# Autodesk Inventor assembly: CartesianRobotWorkSpace
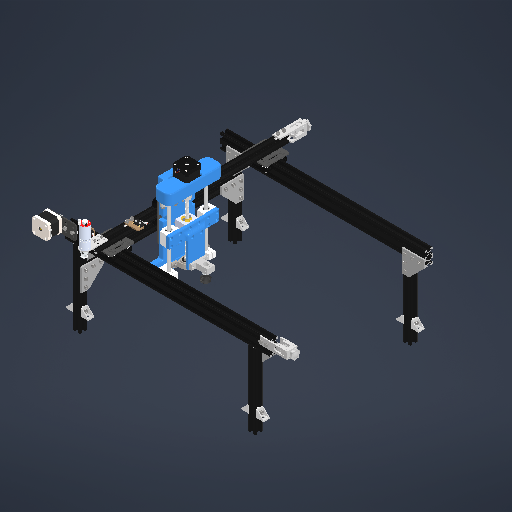
[picture p0: Inventor's stored thumbnail of the model, 512x512]
Saved by Autodesk Inventor 2027.1 (Build 311270010, 270A)
## iProperties
Created: 2026-09-29
Part Number: CartesianRobotWorkSpace
Document SubType Name: Assembly
Designer: SDS Scholar
Author: SDS Scholar
## Documents named in this file (24)
- E:\Apps\AutodeskInventor\University\MCT333_Design_of_Mechatronics_Systems_1\CAD\cartesian_robot_workspace\CartesianRobotWorkSpace.iam
- E:\Apps\AutodeskInventor\University\MCT333_Design_of_Mechatronics_Systems_1\CAD\off_the_shelf_components\AluminiumExtrusion\AluminiumExtrusion2020\Pillars.ipt
- E:\Apps\AutodeskInventor\University\MCT333_Design_of_Mechatronics_Systems_1\CAD\off_the_shelf_components\CornerBracket2020\CornerBracket2020.ipt
- C:\Users\SDS Scholar\Documents\Inventor\Content Center Files\R2027\en-US\SS-ISO 4762\ISO 4762 - M5 x 10SS-ISO.ipt
- E:\Apps\AutodeskInventor\University\MCT333_Design_of_Mechatronics_Systems_1\CAD\off_the_shelf_components\T_nuts\Slider T-Nut for 2020 - M5.ipt
- E:\Apps\AutodeskInventor\University\MCT333_Design_of_Mechatronics_Systems_1\CAD\off_the_shelf_components\RightAngleCornerPlate2020\2020 corner joining plate v1.ipt
- E:\Apps\AutodeskInventor\University\MCT333_Design_of_Mechatronics_Systems_1\CAD\off_the_shelf_components\AluminiumExtrusion\Extrusion2040\2040extrusion_ipt\X_Axis.ipt
- E:\Apps\AutodeskInventor\University\MCT333_Design_of_Mechatronics_Systems_1\CAD\off_the_shelf_components\AluminiumExtrusion\AluminiumExtrusion2020\SupportBeam.ipt
- E:\Apps\AutodeskInventor\University\MCT333_Design_of_Mechatronics_Systems_1\CAD\off_the_shelf_components\VSoltGantrySetAllSizes\20mm Gantry Set\20mm Gantry Set.ipt
- E:\Apps\AutodeskInventor\University\MCT333_Design_of_Mechatronics_Systems_1\CAD\off_the_shelf_components\RightAngleCornerPlate2020\2020 corner joining plate v1_MIR2.ipt
- E:\Apps\AutodeskInventor\University\MCT333_Design_of_Mechatronics_Systems_1\CAD\off_the_shelf_components\T_nuts\Slider T-Nut for 2020 - M5_MIR2.ipt
- E:\Apps\AutodeskInventor\University\MCT333_Design_of_Mechatronics_Systems_1\CAD\off_the_shelf_components\nema-17-23-stepper-motor-mounts\NEMA 17 Flat.ipt
- E:\Apps\AutodeskInventor\University\MCT333_Design_of_Mechatronics_Systems_1\CAD\off_the_shelf_components\GT2BeltTensioner\2020 Belt Tensioner G_K.ipt
- E:\Apps\AutodeskInventor\University\MCT333_Design_of_Mechatronics_Systems_1\CAD\cartesian_robot_workspace\Y_Axis.iam
- E:\Apps\AutodeskInventor\University\MCT333_Design_of_Mechatronics_Systems_1\CAD\cartesian_robot_workspace\Z Axis\Z-Axis.iam
- E:\Apps\AutodeskInventor\University\MCT333_Design_of_Mechatronics_Systems_1\CAD\cartesian_robot_workspace\LimitSwitchMountPlate.ipt
- E:\Apps\AutodeskInventor\University\MCT333_Design_of_Mechatronics_Systems_1\CAD\off_the_shelf_components\T_nuts\Slider T-Nut for 2020 - M3.ipt
- E:\Apps\AutodeskInventor\University\MCT333_Design_of_Mechatronics_Systems_1\CAD\electronic_components\NO-NC Bump Switch\NO-NC Bump Switch.ipt
- C:\Users\SDS Scholar\Documents\Inventor\Content Center Files\R2027\en-US\DIN 7985 (H)\DIN 7985 (H) - M2.5x12-H.ipt
- C:\Users\SDS Scholar\Documents\Inventor\Content Center Files\R2027\en-US\ISO 4032(2)\ISO 4032 - M2.5 - ISO.ipt
- C:\Users\SDS Scholar\Documents\Inventor\Content Center Files\R2027\en-US\ISO 7046-1 H(1)\ISO 7046-1 - M3 x 6_ - 4.8 - H - ISO.ipt
- E:\Apps\AutodeskInventor\University\MCT333_Design_of_Mechatronics_Systems_1\CAD\motors_and_actuators\nema17_stepper_motor\Nema17\Nema17.ipt
- E:\Apps\AutodeskInventor\University\MCT333_Design_of_Mechatronics_Systems_1\CAD\off_the_shelf_components\gt2_pulley_6\GT2 Pulley Assembly With Grub Screws\GT2 Pulley Assembly With Grub Screws.ipt
- E:\Apps\AutodeskInventor\University\MCT333_Design_of_Mechatronics_Systems_1\CAD\DESIGN1_CAD_parameters.xlsx
## Components (131 placed, 22 different names)
1. Z-Axis:1 [sub-assembly] — Tangent:9, Tangent:10, Mate:231, Mate:232
2. SupportBeam:1 — Mate:123, Mate:124, Mate:125, Mate:126, Mate:138, Mate:141, Mate:143, Mate:202
3. X_Axis:1 — Mate:32, Mate:33, Mate:34, Mate:35, Mate:36, Mate:37, Mate:48, Mate:49, Mate:56, Mate:59, Flush:3, Tangent:1, Tangent:2, Mate:145, Mate:146, Mate:147, Mate:148, Mate:151, Mate:154, Flush:6, Mate:156, Mate:157, Mate:158, Mate:159, Mate:162, Mate:165, Mate:217, Flush:193, Mate:234, Mate:235, Mate:236, Mate:237, Mate:240, Mate:243, Mate:268, Mate:271, Mate:274
4. X_Axis:2 — Mate:89, Mate:90, Mate:91, Mate:92, Mate:93, Mate:94, Mate:107, Mate:110, Mate:113, Mate:115, Flush:4, Tangent:5, Tangent:6, Mate:225
5. NEMA 17 Flat:1 — Mate:266, Mate:267, Mate:268, Mate:284, Mate:285, Mate:287, Mate:288, Mate:290, Mate:292, Mate:293, Mate:294, Mate:295, Mate:296
6. Slider T-Nut for 2020 - M5:40 — Mate:145, Mate:146, Mate:150, Flush:6
7. Slider T-Nut for 2020 - M5:41 — Mate:147, Mate:148, Mate:153
8. SS ISO 4762 M5 x 10:58 — Mate:150, Mate:151, Mate:270
9. SS ISO 4762 M5 x 10:59 — Mate:153, Mate:154, Mate:269
10. ISO 7046-1 H M3 x 6 - 4.8 - H:1 — Mate:285, Mate:286, Mate:293
11. ISO 7046-1 H M3 x 6 - 4.8 - H:2 — Mate:287, Mate:294
12. ISO 7046-1 H M3 x 6 - 4.8 - H:3 — Mate:288, Mate:289, Mate:292
13. Nema17:1 — Mate:284, Mate:286, Mate:289, Mate:291, Mate:296, Mate:297, Mate:298
14. ISO 7046-1 H M3 x 6 - 4.8 - H:4 — Mate:290, Mate:291, Mate:295
15. GT2 Pulley Assembly With Grub Screws:1 — Mate:297, Mate:298
16. 2020 Belt Tensioner G_K:1 — Mate:269, Mate:270, Mate:271
17. Slider T-Nut for 2020 - M5:42 — Mate:156, Mate:157, Mate:161, Mate:179, Flush:193
18. Slider T-Nut for 2020 - M5:43 — Mate:158, Mate:159, Mate:164
19. SS ISO 4762 M5 x 10:60 — Mate:164, Mate:165, Mate:266
20. SS ISO 4762 M5 x 10:61 — Mate:161, Mate:162, Mate:179, Mate:267
21. 20mm Gantry Set:1 — Tangent:1, Tangent:2, Flush:5, Mate:171, Flush:9, Mate:229, Mate:230
22. 20mm Gantry Set:2 — Tangent:5, Tangent:6, Flush:5, Mate:174, Mate:177, Flush:8, Flush:9
23. Y_Axis:1 [sub-assembly] — Mate:167, Mate:168, Mate:169, Mate:170, Mate:173, Mate:176, Mate:177, Flush:8, Tangent:9, Tangent:10, Mate:231, Mate:232
24. Slider T-Nut for 2020 - M5:44 — Mate:167, Mate:168, Mate:172
25. Slider T-Nut for 2020 - M5:45 — Mate:169, Mate:170, Mate:175
26. SS ISO 4762 M5 x 10:62 — Mate:174, Mate:175, Mate:176
27. SS ISO 4762 M5 x 10:63 — Mate:171, Mate:172, Mate:173
28. NO-NC Bump Switch:1 — Mate:279, Mate:280, Mate:281, Mate:282, Mate:283
29. LimitSwitchMountPlate:1 — Mate:272, Mate:273, Mate:274, Flush:194, Mate:275, Mate:276, Mate:277, Mate:278, Mate:281
30. Slider T-Nut for 2020 - M3:1 — Mate:234, Mate:235, Mate:239
31. Slider T-Nut for 2020 - M3:2 — Mate:236, Mate:237, Mate:242
32. SS ISO 4762 M5 x 10:70 — Mate:239, Mate:240, Mate:273
33. SS ISO 4762 M5 x 10:71 — Mate:242, Mate:243, Mate:272
34. DIN 7985 (H) M2.5x12-H:1 — Mate:251, Mate:275, Mate:279, Mate:282
35. DIN 7985 (H) M2.5x12-H:2 — Mate:253, Mate:276, Mate:280, Mate:283
36. ISO 4032 M2.5:1 — Mate:251, Mate:277
37. ISO 4032 M2.5:2 — Mate:253, Mate:278
38. Pillars:1 — Flush:10, Flush:11, Mate:183, Mate:184, Mate:185, Mate:186, Mate:187, Mate:188, Mate:189, Flush:191, Flush:192, Mate:190, Symmetry:1, Mate:191, Mate:192, Mate:193, Mate:194, Mate:195, Mate:196, Mate:197, Mate:198, Mate:199, Mate:200, Mate:201, Mate:202
39. SS ISO 4762 M5 x 10:2 — Mate:28, Mate:29, Mate:189
40. Slider T-Nut for 2020 - M5:2 — Mate:29, Mate:186, Mate:187
41. Slider T-Nut for 2020 - M5:1 — Mate:21, Mate:184, Mate:185
42. SS ISO 4762 M5 x 10:1 — Mate:20, Mate:21, Mate:31, Mate:188
43. CornerBracket2020:1 — Mate:20, Mate:31, Flush:191
44. CornerBracket2020:4 — Mate:28, Flush:192, Mate:190
45. Pillars:2 — Mate:218, Mate:219, Mate:220, Mate:221, Mate:222, Mate:223, Mate:224, Mate:225
46. SS ISO 4762 M5 x 10:64
47. Slider T-Nut for 2020 - M5:46
48. Slider T-Nut for 2020 - M5:47
49. SS ISO 4762 M5 x 10:65
50. CornerBracket2020:5
51. CornerBracket2020:6
52. Pillars:3 — Symmetry:1
53. SS ISO 4762 M5 x 10:66
54. Slider T-Nut for 2020 - M5:48
55. Slider T-Nut for 2020 - M5:49
56. SS ISO 4762 M5 x 10:67
57. CornerBracket2020:7
58. CornerBracket2020:8
59. Pillars:4 — Mate:210, Mate:211, Mate:212, Mate:213, Mate:214, Mate:215, Mate:216, Mate:217
60. SS ISO 4762 M5 x 10:68
61. Slider T-Nut for 2020 - M5:50
62. Slider T-Nut for 2020 - M5:51
63. SS ISO 4762 M5 x 10:69
64. CornerBracket2020:9
65. CornerBracket2020:10
66. 2020 corner joining plate v1:6 — Mate:127, Mate:130, Mate:133, Mate:136, Mate:139, Mate:143, Mate:144, Mate:201
67. Slider T-Nut for 2020 - M5:35 — Mate:131, Mate:192, Mate:195
68. Slider T-Nut for 2020 - M5:36 — Mate:123, Mate:124, Mate:137
69. Slider T-Nut for 2020 - M5:37 — Mate:134, Mate:191, Mate:194, Mate:196
70. Slider T-Nut for 2020 - M5:38 — Mate:125, Mate:126, Mate:140
71. Slider T-Nut for 2020 - M5:39 — Mate:128, Mate:193, Mate:197
72. SS ISO 4762 M5 x 10:48 — Mate:127, Mate:128, Mate:198
73. SS ISO 4762 M5 x 10:49 — Mate:139, Mate:140, Mate:141
74. SS ISO 4762 M5 x 10:50 — Mate:130, Mate:131, Mate:199
75. SS ISO 4762 M5 x 10:51 — Mate:133, Mate:134, Mate:200
76. SS ISO 4762 M5 x 10:52 — Mate:136, Mate:137, Mate:138
77. 2020 corner joining plate v1_MIR2:1
78. Slider T-Nut for 2020 - M5_MIR2:1
79. Slider T-Nut for 2020 - M5_MIR2:2
80. Slider T-Nut for 2020 - M5_MIR2:3
81. Slider T-Nut for 2020 - M5_MIR2:4
82. Slider T-Nut for 2020 - M5_MIR2:5
83. SS ISO 4762 M5 x 10:53
84. SS ISO 4762 M5 x 10:54
85. SS ISO 4762 M5 x 10:55
86. SS ISO 4762 M5 x 10:56
87. SS ISO 4762 M5 x 10:57
88. 2020 corner joining plate v1:1 — Mate:42, Mate:46, Mate:49, Mate:51, Mate:54, Mate:57, Flush:3, Mate:216, Mate:230
89. Slider T-Nut for 2020 - M5:9 — Mate:36, Mate:37, Mate:55
90. Slider T-Nut for 2020 - M5:10 — Mate:52, Mate:212, Mate:213
91. Slider T-Nut for 2020 - M5:11 — Mate:43, Mate:210, Mate:211
92. Slider T-Nut for 2020 - M5:12 — Mate:34, Mate:35, Mate:58
93. Slider T-Nut for 2020 - M5:13 — Mate:32, Mate:33, Mate:47
94. SS ISO 4762 M5 x 10:9 — Mate:42, Mate:43, Mate:215
95. SS ISO 4762 M5 x 10:10 — Mate:46, Mate:47, Mate:48
96. SS ISO 4762 M5 x 10:11 — Mate:54, Mate:55, Mate:56
97. SS ISO 4762 M5 x 10:12 — Mate:51, Mate:52, Mate:214
98. SS ISO 4762 M5 x 10:13 — Mate:57, Mate:58, Mate:59
99. 2020 corner joining plate v1:2 — Mate:229, Flush:194
100. Slider T-Nut for 2020 - M5:14
101. Slider T-Nut for 2020 - M5:15
102. Slider T-Nut for 2020 - M5:16
103. Slider T-Nut for 2020 - M5:17
104. Slider T-Nut for 2020 - M5:18
105. SS ISO 4762 M5 x 10:14
106. SS ISO 4762 M5 x 10:15
107. SS ISO 4762 M5 x 10:16
108. SS ISO 4762 M5 x 10:17
109. SS ISO 4762 M5 x 10:18
110. 2020 corner joining plate v1:4 — Mate:99, Mate:102, Mate:105, Mate:108, Mate:111, Mate:115, Flush:4, Mate:224
111. Slider T-Nut for 2020 - M5:25 — Mate:93, Mate:94, Mate:106
112. Slider T-Nut for 2020 - M5:26 — Mate:103, Mate:218, Mate:219
113. Slider T-Nut for 2020 - M5:27 — Mate:100, Mate:220, Mate:221
114. Slider T-Nut for 2020 - M5:28 — Mate:91, Mate:92, Mate:109
115. Slider T-Nut for 2020 - M5:29 — Mate:89, Mate:90, Mate:112
116. SS ISO 4762 M5 x 10:38 — Mate:99, Mate:100, Mate:223
117. SS ISO 4762 M5 x 10:39 — Mate:105, Mate:106, Mate:107
118. SS ISO 4762 M5 x 10:40 — Mate:102, Mate:103, Mate:222
119. SS ISO 4762 M5 x 10:41 — Mate:108, Mate:109, Mate:110
120. SS ISO 4762 M5 x 10:42 — Mate:111, Mate:112, Mate:113
121. 2020 corner joining plate v1:5 — Mate:144
122. Slider T-Nut for 2020 - M5:30
123. Slider T-Nut for 2020 - M5:31
124. Slider T-Nut for 2020 - M5:32
125. Slider T-Nut for 2020 - M5:33
126. Slider T-Nut for 2020 - M5:34
127. SS ISO 4762 M5 x 10:43
128. SS ISO 4762 M5 x 10:44
129. SS ISO 4762 M5 x 10:45
130. SS ISO 4762 M5 x 10:46
131. SS ISO 4762 M5 x 10:47
## Component patterns: (4 elements, first: Pillars:1 + SS ISO 4762 M5 x 10:2 + Slider T-Nut for 2020 - M5:2 + Slider T-Nut for 2020 - M5:1 + SS ISO 4762 M5 x 10:1 + CornerBracket2020:1 + CornerBracket2020:4), (2 elements, first: 2020 corner joining plate v1:6 + Slider T-Nut for 2020 - M5:35 + Slider T-Nut for 2020 - M5:36 + Slider T-Nut for 2020 - M5:37 + Slider T-Nut for 2020 - M5:38 + Slider T-Nut for 2020 - M5:39 + SS ISO 4762 M5 x 10:48 + SS ISO 4762 M5 x 10:49 + SS ISO 4762 M5 x 10:50 + SS ISO 4762 M5 x 10:51 + SS ISO 4762 M5 x 10:52), (2 elements, first: 2020 corner joining plate v1:1 + Slider T-Nut for 2020 - M5:9 + Slider T-Nut for 2020 - M5:10 + Slider T-Nut for 2020 - M5:11 + Slider T-Nut for 2020 - M5:12 + Slider T-Nut for 2020 - M5:13 + SS ISO 4762 M5 x 10:9 + SS ISO 4762 M5 x 10:10 + SS ISO 4762 M5 x 10:11 + SS ISO 4762 M5 x 10:12 + SS ISO 4762 M5 x 10:13), (2 elements, first: 2020 corner joining plate v1:4 + Slider T-Nut for 2020 - M5:25 + Slider T-Nut for 2020 - M5:26 + Slider T-Nut for 2020 - M5:27 + Slider T-Nut for 2020 - M5:28 + Slider T-Nut for 2020 - M5:29 + SS ISO 4762 M5 x 10:38 + SS ISO 4762 M5 x 10:39 + SS ISO 4762 M5 x 10:40 + SS ISO 4762 M5 x 10:41 + SS ISO 4762 M5 x 10:42)
## Relationships (193: Mate 174, Flush 12, Tangent 6, Symmetry 1)
- Mate:20: SS ISO 4762 M5 x 10:1 ↔ CornerBracket2020:1
- Mate:21: Slider T-Nut for 2020 - M5:1 ↔ SS ISO 4762 M5 x 10:1
- Mate:28: SS ISO 4762 M5 x 10:2 ↔ CornerBracket2020:4
- Mate:29: SS ISO 4762 M5 x 10:2 ↔ Slider T-Nut for 2020 - M5:2
- Mate:31 (0.7 mm): SS ISO 4762 M5 x 10:1 ↔ CornerBracket2020:1
- Mate:32: X_Axis:1 ↔ Slider T-Nut for 2020 - M5:13
- Mate:33: X_Axis:1 ↔ Slider T-Nut for 2020 - M5:13
- Mate:34: X_Axis:1 ↔ Slider T-Nut for 2020 - M5:12
- Mate:35: X_Axis:1 ↔ Slider T-Nut for 2020 - M5:12
- Mate:36: X_Axis:1 ↔ Slider T-Nut for 2020 - M5:9
- Mate:37: X_Axis:1 ↔ Slider T-Nut for 2020 - M5:9
- Mate:42: 2020 corner joining plate v1:1 ↔ SS ISO 4762 M5 x 10:9
- Mate:43: Slider T-Nut for 2020 - M5:11 ↔ SS ISO 4762 M5 x 10:9
- Mate:46: 2020 corner joining plate v1:1 ↔ SS ISO 4762 M5 x 10:10
- Mate:47: Slider T-Nut for 2020 - M5:13 ↔ SS ISO 4762 M5 x 10:10
- Mate:48: X_Axis:1 ↔ SS ISO 4762 M5 x 10:10
- Mate:49: X_Axis:1 ↔ 2020 corner joining plate v1:1
- Mate:51: 2020 corner joining plate v1:1 ↔ SS ISO 4762 M5 x 10:12
- Mate:52: Slider T-Nut for 2020 - M5:10 ↔ SS ISO 4762 M5 x 10:12
- Mate:54: 2020 corner joining plate v1:1 ↔ SS ISO 4762 M5 x 10:11
- Mate:55: Slider T-Nut for 2020 - M5:9 ↔ SS ISO 4762 M5 x 10:11
- Mate:56: X_Axis:1 ↔ SS ISO 4762 M5 x 10:11
- Mate:57: 2020 corner joining plate v1:1 ↔ SS ISO 4762 M5 x 10:13
- Mate:58: Slider T-Nut for 2020 - M5:12 ↔ SS ISO 4762 M5 x 10:13
- Mate:59: X_Axis:1 ↔ SS ISO 4762 M5 x 10:13
- Flush:3: X_Axis:1 ↔ 2020 corner joining plate v1:1
- Tangent:1: X_Axis:1 ↔ 20mm Gantry Set:1
- Tangent:2: X_Axis:1 ↔ 20mm Gantry Set:1
- Mate:89: X_Axis:2 ↔ Slider T-Nut for 2020 - M5:29
- Mate:90: X_Axis:2 ↔ Slider T-Nut for 2020 - M5:29
- Mate:91: X_Axis:2 ↔ Slider T-Nut for 2020 - M5:28
- Mate:92: X_Axis:2 ↔ Slider T-Nut for 2020 - M5:28
- Mate:93: X_Axis:2 ↔ Slider T-Nut for 2020 - M5:25
- Mate:94: X_Axis:2 ↔ Slider T-Nut for 2020 - M5:25
- Mate:99: 2020 corner joining plate v1:4 ↔ SS ISO 4762 M5 x 10:38
- Mate:100: Slider T-Nut for 2020 - M5:27 ↔ SS ISO 4762 M5 x 10:38
- Mate:102: 2020 corner joining plate v1:4 ↔ SS ISO 4762 M5 x 10:40
- Mate:103: Slider T-Nut for 2020 - M5:26 ↔ SS ISO 4762 M5 x 10:40
- Mate:105: 2020 corner joining plate v1:4 ↔ SS ISO 4762 M5 x 10:39
- Mate:106: Slider T-Nut for 2020 - M5:25 ↔ SS ISO 4762 M5 x 10:39
- Mate:107: X_Axis:2 ↔ SS ISO 4762 M5 x 10:39
- Mate:108: 2020 corner joining plate v1:4 ↔ SS ISO 4762 M5 x 10:41
- Mate:109: Slider T-Nut for 2020 - M5:28 ↔ SS ISO 4762 M5 x 10:41
- Mate:110: X_Axis:2 ↔ SS ISO 4762 M5 x 10:41
- Mate:111: 2020 corner joining plate v1:4 ↔ SS ISO 4762 M5 x 10:42
- Mate:112: Slider T-Nut for 2020 - M5:29 ↔ SS ISO 4762 M5 x 10:42
- Mate:113: X_Axis:2 ↔ SS ISO 4762 M5 x 10:42
- Mate:115: X_Axis:2 ↔ 2020 corner joining plate v1:4
- Flush:4: X_Axis:2 ↔ 2020 corner joining plate v1:4
- Mate:123: SupportBeam:1 ↔ Slider T-Nut for 2020 - M5:36
- Mate:124: SupportBeam:1 ↔ Slider T-Nut for 2020 - M5:36
- Mate:125: SupportBeam:1 ↔ Slider T-Nut for 2020 - M5:38
- Mate:126: SupportBeam:1 ↔ Slider T-Nut for 2020 - M5:38
- Mate:127: 2020 corner joining plate v1:6 ↔ SS ISO 4762 M5 x 10:48
- Mate:128: Slider T-Nut for 2020 - M5:39 ↔ SS ISO 4762 M5 x 10:48
- Mate:130: 2020 corner joining plate v1:6 ↔ SS ISO 4762 M5 x 10:50
- Mate:131: Slider T-Nut for 2020 - M5:35 ↔ SS ISO 4762 M5 x 10:50
- Mate:133: 2020 corner joining plate v1:6 ↔ SS ISO 4762 M5 x 10:51
- Mate:134: Slider T-Nut for 2020 - M5:37 ↔ SS ISO 4762 M5 x 10:51
- Mate:136: 2020 corner joining plate v1:6 ↔ SS ISO 4762 M5 x 10:52
- Mate:137: Slider T-Nut for 2020 - M5:36 ↔ SS ISO 4762 M5 x 10:52
- Mate:138: SupportBeam:1 ↔ SS ISO 4762 M5 x 10:52
- Mate:139: 2020 corner joining plate v1:6 ↔ SS ISO 4762 M5 x 10:49
- Mate:140: Slider T-Nut for 2020 - M5:38 ↔ SS ISO 4762 M5 x 10:49
- Mate:141: SupportBeam:1 ↔ SS ISO 4762 M5 x 10:49
- Mate:143: SupportBeam:1 ↔ 2020 corner joining plate v1:6
- Mate:144 (5 mm): 2020 corner joining plate v1:6 ↔ 2020 corner joining plate v1:5
- Tangent:5: X_Axis:2 ↔ 20mm Gantry Set:2
- Tangent:6: X_Axis:2 ↔ 20mm Gantry Set:2
- Flush:5: 20mm Gantry Set:1 ↔ 20mm Gantry Set:2
- Mate:145: X_Axis:1 ↔ Slider T-Nut for 2020 - M5:40
- Mate:146: X_Axis:1 ↔ Slider T-Nut for 2020 - M5:40
- Mate:147: X_Axis:1 ↔ Slider T-Nut for 2020 - M5:41
- Mate:148: X_Axis:1 ↔ Slider T-Nut for 2020 - M5:41
- Mate:150: Slider T-Nut for 2020 - M5:40 ↔ SS ISO 4762 M5 x 10:58
- Mate:151: X_Axis:1 ↔ SS ISO 4762 M5 x 10:58
- Mate:153: Slider T-Nut for 2020 - M5:41 ↔ SS ISO 4762 M5 x 10:59
- Mate:154: X_Axis:1 ↔ SS ISO 4762 M5 x 10:59
- Flush:6: X_Axis:1 ↔ Slider T-Nut for 2020 - M5:40
- Mate:156: X_Axis:1 ↔ Slider T-Nut for 2020 - M5:42
- Mate:157: X_Axis:1 ↔ Slider T-Nut for 2020 - M5:42
- Mate:158: X_Axis:1 ↔ Slider T-Nut for 2020 - M5:43
- Mate:159: X_Axis:1 ↔ Slider T-Nut for 2020 - M5:43
- Mate:161: Slider T-Nut for 2020 - M5:42 ↔ SS ISO 4762 M5 x 10:61
- Mate:162: X_Axis:1 ↔ SS ISO 4762 M5 x 10:61
- Mate:164: Slider T-Nut for 2020 - M5:43 ↔ SS ISO 4762 M5 x 10:60
- Mate:165: X_Axis:1 ↔ SS ISO 4762 M5 x 10:60
- Mate:167: Y_Axis:1 ↔ Slider T-Nut for 2020 - M5:44
- Mate:168: Y_Axis:1 ↔ Slider T-Nut for 2020 - M5:44
- Mate:169: Y_Axis:1 ↔ Slider T-Nut for 2020 - M5:45
- Mate:170: Y_Axis:1 ↔ Slider T-Nut for 2020 - M5:45
- Mate:171: 20mm Gantry Set:1 ↔ SS ISO 4762 M5 x 10:63
- Mate:172: Slider T-Nut for 2020 - M5:44 ↔ SS ISO 4762 M5 x 10:63
- Mate:173: Y_Axis:1 ↔ SS ISO 4762 M5 x 10:63
- Mate:174: 20mm Gantry Set:2 ↔ SS ISO 4762 M5 x 10:62
- Mate:175: Slider T-Nut for 2020 - M5:45 ↔ SS ISO 4762 M5 x 10:62
- Mate:176: Y_Axis:1 ↔ SS ISO 4762 M5 x 10:62
- Mate:177: 20mm Gantry Set:2 ↔ Y_Axis:1
- Flush:8 (-20 mm): 20mm Gantry Set:2 ↔ Y_Axis:1
- Flush:9: 20mm Gantry Set:1 ↔ 20mm Gantry Set:2
- Mate:179: Slider T-Nut for 2020 - M5:42 ↔ SS ISO 4762 M5 x 10:61
- Flush:10: Pillars:1
- Flush:11: Pillars:1
- Mate:183: Pillars:1
- Mate:184: Pillars:1 ↔ Slider T-Nut for 2020 - M5:1
- Mate:185: Pillars:1 ↔ Slider T-Nut for 2020 - M5:1
- Mate:186: Pillars:1 ↔ Slider T-Nut for 2020 - M5:2
- Mate:187: Pillars:1 ↔ Slider T-Nut for 2020 - M5:2
- Mate:188: Pillars:1 ↔ SS ISO 4762 M5 x 10:1
- Mate:189: Pillars:1 ↔ SS ISO 4762 M5 x 10:2
- Flush:191 (40 mm): Pillars:1 ↔ CornerBracket2020:1
- Flush:192 (40 mm): Pillars:1 ↔ CornerBracket2020:4
- Mate:190: Pillars:1 ↔ CornerBracket2020:4
- Symmetry:1: Pillars:1 ↔ Pillars:3
- Mate:191: Pillars:1 ↔ Slider T-Nut for 2020 - M5:37
- Mate:192: Pillars:1 ↔ Slider T-Nut for 2020 - M5:35
- Mate:193: Pillars:1 ↔ Slider T-Nut for 2020 - M5:39
- Mate:194: Pillars:1 ↔ Slider T-Nut for 2020 - M5:37
- Mate:195: Pillars:1 ↔ Slider T-Nut for 2020 - M5:35
- Mate:196: Pillars:1 ↔ Slider T-Nut for 2020 - M5:37
- Mate:197: Pillars:1 ↔ Slider T-Nut for 2020 - M5:39
- Mate:198: Pillars:1 ↔ SS ISO 4762 M5 x 10:48
- Mate:199: Pillars:1 ↔ SS ISO 4762 M5 x 10:50
- Mate:200: Pillars:1 ↔ SS ISO 4762 M5 x 10:51
- Mate:201: Pillars:1 ↔ 2020 corner joining plate v1:6
- Mate:202: SupportBeam:1 ↔ Pillars:1
- Mate:210: Pillars:4 ↔ Slider T-Nut for 2020 - M5:11
- Mate:211: Pillars:4 ↔ Slider T-Nut for 2020 - M5:11
- Mate:212: Pillars:4 ↔ Slider T-Nut for 2020 - M5:10
- Mate:213: Pillars:4 ↔ Slider T-Nut for 2020 - M5:10
- Mate:214: Pillars:4 ↔ SS ISO 4762 M5 x 10:12
- Mate:215: Pillars:4 ↔ SS ISO 4762 M5 x 10:9
- Mate:216: Pillars:4 ↔ 2020 corner joining plate v1:1
- Mate:217: X_Axis:1 ↔ Pillars:4
- Mate:218: Pillars:2 ↔ Slider T-Nut for 2020 - M5:26
- Mate:219: Pillars:2 ↔ Slider T-Nut for 2020 - M5:26
- Mate:220: Pillars:2 ↔ Slider T-Nut for 2020 - M5:27
- Mate:221: Pillars:2 ↔ Slider T-Nut for 2020 - M5:27
- Mate:222: Pillars:2 ↔ SS ISO 4762 M5 x 10:40
- Mate:223: Pillars:2 ↔ SS ISO 4762 M5 x 10:38
- Mate:224: Pillars:2 ↔ 2020 corner joining plate v1:4
- Mate:225: X_Axis:2 ↔ Pillars:2
- Flush:193: X_Axis:1 ↔ Slider T-Nut for 2020 - M5:42
- Tangent:9: Z-Axis:1 ↔ Y_Axis:1
- Tangent:10: Z-Axis:1 ↔ Y_Axis:1
- Mate:229: 20mm Gantry Set:1 ↔ 2020 corner joining plate v1:2
- Mate:230: 20mm Gantry Set:1 ↔ 2020 corner joining plate v1:1
- Mate:231: Z-Axis:1 ↔ Y_Axis:1
- Mate:232: Z-Axis:1 ↔ Y_Axis:1
- Mate:234: X_Axis:1 ↔ Slider T-Nut for 2020 - M3:1
- Mate:235: X_Axis:1 ↔ Slider T-Nut for 2020 - M3:1
- Mate:236: X_Axis:1 ↔ Slider T-Nut for 2020 - M3:2
- Mate:237: X_Axis:1 ↔ Slider T-Nut for 2020 - M3:2
- Mate:239: Slider T-Nut for 2020 - M3:1 ↔ SS ISO 4762 M5 x 10:70
- Mate:240: X_Axis:1 ↔ SS ISO 4762 M5 x 10:70
- Mate:242: Slider T-Nut for 2020 - M3:2 ↔ SS ISO 4762 M5 x 10:71
- Mate:243: X_Axis:1 ↔ SS ISO 4762 M5 x 10:71
- Mate:251: DIN 7985 (H) M2.5x12-H:1 ↔ ISO 4032 M2.5:1
- Mate:253: DIN 7985 (H) M2.5x12-H:2 ↔ ISO 4032 M2.5:2
- Mate:266: NEMA 17 Flat:1 ↔ SS ISO 4762 M5 x 10:60
- Mate:267: NEMA 17 Flat:1 ↔ SS ISO 4762 M5 x 10:61
- Mate:268: X_Axis:1 ↔ NEMA 17 Flat:1
- Mate:269: SS ISO 4762 M5 x 10:59 ↔ 2020 Belt Tensioner G_K:1
- Mate:270: SS ISO 4762 M5 x 10:58 ↔ 2020 Belt Tensioner G_K:1
- Mate:271: X_Axis:1 ↔ 2020 Belt Tensioner G_K:1
- Mate:272: LimitSwitchMountPlate:1 ↔ SS ISO 4762 M5 x 10:71
- Mate:273: LimitSwitchMountPlate:1 ↔ SS ISO 4762 M5 x 10:70
- Mate:274: X_Axis:1 ↔ LimitSwitchMountPlate:1
- Flush:194: LimitSwitchMountPlate:1 ↔ 2020 corner joining plate v1:2
- Mate:275: LimitSwitchMountPlate:1 ↔ DIN 7985 (H) M2.5x12-H:1
- Mate:276: LimitSwitchMountPlate:1 ↔ DIN 7985 (H) M2.5x12-H:2
- Mate:277: LimitSwitchMountPlate:1 ↔ ISO 4032 M2.5:1
- Mate:278: LimitSwitchMountPlate:1 ↔ ISO 4032 M2.5:2
- Mate:279: NO-NC Bump Switch:1 ↔ DIN 7985 (H) M2.5x12-H:1
- Mate:280: NO-NC Bump Switch:1 ↔ DIN 7985 (H) M2.5x12-H:2
- Mate:281: NO-NC Bump Switch:1 ↔ LimitSwitchMountPlate:1
- Mate:282: NO-NC Bump Switch:1 ↔ DIN 7985 (H) M2.5x12-H:1
- Mate:283: NO-NC Bump Switch:1 ↔ DIN 7985 (H) M2.5x12-H:2
- Mate:284: NEMA 17 Flat:1 ↔ Nema17:1
- Mate:285: NEMA 17 Flat:1 ↔ ISO 7046-1 H M3 x 6 - 4.8 - H:1
- Mate:286: ISO 7046-1 H M3 x 6 - 4.8 - H:1 ↔ Nema17:1
- Mate:287: NEMA 17 Flat:1 ↔ ISO 7046-1 H M3 x 6 - 4.8 - H:2
- Mate:288: NEMA 17 Flat:1 ↔ ISO 7046-1 H M3 x 6 - 4.8 - H:3
- Mate:289: ISO 7046-1 H M3 x 6 - 4.8 - H:3 ↔ Nema17:1
- Mate:290: NEMA 17 Flat:1 ↔ ISO 7046-1 H M3 x 6 - 4.8 - H:4
- Mate:291: Nema17:1 ↔ ISO 7046-1 H M3 x 6 - 4.8 - H:4
- Mate:292: NEMA 17 Flat:1 ↔ ISO 7046-1 H M3 x 6 - 4.8 - H:3
- Mate:293: NEMA 17 Flat:1 ↔ ISO 7046-1 H M3 x 6 - 4.8 - H:1
- Mate:294: NEMA 17 Flat:1 ↔ ISO 7046-1 H M3 x 6 - 4.8 - H:2
- Mate:295: NEMA 17 Flat:1 ↔ ISO 7046-1 H M3 x 6 - 4.8 - H:4
- Mate:296: NEMA 17 Flat:1 ↔ Nema17:1
- Mate:297: Nema17:1 ↔ GT2 Pulley Assembly With Grub Screws:1
- Mate:298: Nema17:1 ↔ GT2 Pulley Assembly With Grub Screws:1
## Named parameters: Product_dia = 50 mm, ProductBaseHeight = 40 mm, ProductLedHeight = 20 mm, GridProcutClearance = 3 mm, GridBorderThickness = 5 mm, GridBorderFillets = 7 mm, GridTotalSize = 63 mm, GridRobotClearance = 50 mm, AluminiumExtrusionBase = 20 mm, AluminiumExtrusionClearance = 30 mm, BaseTotalWidth = 652 mm, FeedingAreaLength = 400 mm, BaseTotalLength = 912 mm, DistanceBetweenGrid = 5 mm, WorkspaceLength = 552 mm, WorkspaceWidth = 417 mm, WorkspaceHeight = 136.5 mm, AxesBaseFillet = 15 mm, Zaxis = 223 mm, ProductTotalHeight = 45 mm, VerticalClearance = 10 mm, VerticalStroke = 85 mm, FrontArea = 50 mm, BackArea = 150 mm, CylinderStroke = 75 mm, SideAreaWidth = 200 mm, BaseHeight = 70 mm, ContolBoxLength = 100 mm, DistanceBetweenBoxes = 30 mm, BoxesWidth = 140 mm, PowerBoxLength = 630 mm, PneumaticBoxLength = 200 mm, BoxesClearance = 30 mm, BoxesHeight = 70 mm, ContolBoxWidth = 200 mm, ControlBoxHeight = 70 mm, BaseWoodThickness = 7 mm, kerf = 1.5 mm, Kerf = 0.3 mm, TransmitterAreaWidth = 100 mm, RxThickness = 1.8 mm
